# Autodesk Inventor assembly: EnsambleConexionesSalidas
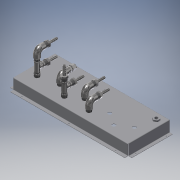
[picture p0: Inventor's stored thumbnail of the model, 180x180]
Saved by Autodesk Inventor 2017 (Build 210142000, 142)
## iProperties
Created: 2021-06-29
Part Number: EnsambleConexionesSalidas
Document SubType Name: Assembly
Designer: USUARIO
Author: USUARIO
## Documents named in this file (8)
- D:\Laboratorio\Autoclave\Autoclave Horizontal\Con Precamara\2021\Autoclave 110L Biocacol OP2021110 #0045886XX\Modelo\Planos\EnsambleConexionesSalidas.iam
- D:\Laboratorio\Autoclave\Autoclave Horizontal\Con Precamara\2021\Autoclave 110L Biocacol OP2021110 #0045886XX\Modelo\COMPLEMENTO POSTERIOR ACH-110L-2021-P.ipt
- C:\Modelos 3D y DXF\Racores\B3 1-2x1-2.ipt
- C:\Modelos 3D y DXF\Racores\User Library-Tee_Class300.ipt
- C:\Modelos 3D y DXF\Racores\User Library-codo a 90 de 1-2-Rosc.ipt
- C:\Modelos 3D y DXF\Racores\1-2-1-2-SwagelokCompany-3D-06-16-2021.ipt
- C:\Modelos 3D y DXF\Racores\CodoCalle.iam
- C:\Modelos 3D y DXF\Prensacables\User Library-BUD CABLE GLAND.ipt
## Components (20 placed, 7 different names)
1. COMPLEMENTO POSTERIOR ACH-110L-2021-P:1
2. B3 1-2x1-2:1
3. User Library-Tee_Class300:1
4. B3 1-2x1-2:2
5. B3 1-2x1-2:3
6. B3 1-2x1-2:4
7. B3 1-2x1-2:5
8. User Library-Tee_Class300:2
9. B3 1-2x1-2:6
10. B3 1-2x1-2:7
11. User Library-codo a 90 de 1-2-Rosc:1
12. B3 1-2x1-2:8
13. User Library-codo a 90 de 1-2-Rosc:2
14. B3 1-2x1-2:9
15. B3 1-2x1-2:10
16. 1-2-1-2-SwagelokCompany-3D-06-16-2021:1
17. User Library-codo a 90 de 1-2-Rosc:3
18. CodoCalle:1 [sub-assembly]
19. B3 1-2x1-2:11
20. User Library-BUD CABLE GLAND:1
## Relationships (19: Insert 19)
- [Insert]: COMPLEMENTO POSTERIOR ACH-110L-2021-P:1 ↔ B3 1-2x1-2:1
- [Insert] (-9 mm): B3 1-2x1-2:1 ↔ User Library-Tee_Class300:1
- [Insert] (-9 mm): User Library-Tee_Class300:1 ↔ B3 1-2x1-2:2
- [Insert] (-9 mm): User Library-Tee_Class300:1 ↔ B3 1-2x1-2:3
- [Insert]: COMPLEMENTO POSTERIOR ACH-110L-2021-P:1 ↔ B3 1-2x1-2:4
- [Insert]: COMPLEMENTO POSTERIOR ACH-110L-2021-P:1 ↔ B3 1-2x1-2:5
- [Insert] (-9 mm): User Library-Tee_Class300:2 ↔ B3 1-2x1-2:6
- [Insert] (10 mm): B3 1-2x1-2:5 ↔ User Library-Tee_Class300:2
- [Insert]: COMPLEMENTO POSTERIOR ACH-110L-2021-P:1 ↔ B3 1-2x1-2:7
- [Insert] (-9 mm): User Library-codo a 90 de 1-2-Rosc:1 ↔ B3 1-2x1-2:8
- [Insert] (-9 mm): User Library-codo a 90 de 1-2-Rosc:2 ↔ B3 1-2x1-2:9
- [Insert] (-9 mm): B3 1-2x1-2:7 ↔ User Library-codo a 90 de 1-2-Rosc:1
- [Insert]: COMPLEMENTO POSTERIOR ACH-110L-2021-P:1 ↔ B3 1-2x1-2:10
- [Insert] (-9 mm): User Library-codo a 90 de 1-2-Rosc:2 ↔ B3 1-2x1-2:10
- [Insert] (-9 mm): B3 1-2x1-2:4 ↔ User Library-codo a 90 de 1-2-Rosc:3
- [Insert] (9 mm): 1-2-1-2-SwagelokCompany-3D-06-16-2021:1 ↔ User Library-codo a 90 de 1-2-Rosc:3
- [Insert] (-9 mm): User Library-Tee_Class300:2 ↔ CodoCalle:1
- [Insert] (-9 mm): CodoCalle:1 ↔ B3 1-2x1-2:11
- [Insert]: COMPLEMENTO POSTERIOR ACH-110L-2021-P:1 ↔ User Library-BUD CABLE GLAND:1
## Named parameters: d167_d166 = -9 mm, d148_d141 = -9 mm
